# Autodesk Inventor assembly: BevelGear_Ref
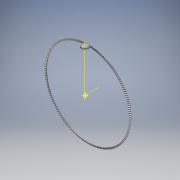
[picture p0: Inventor's stored thumbnail of the model, 180x180]
Saved by Autodesk Inventor 2017 (Build 210142000, 142)
## iProperties
Created: 2017-01-19
Part Number: BevelGear_Ref
Document SubType Name: Assembly
Designer: David Kopala
Author: David Kopala
## Documents named in this file (2)
- Z:\Documents\Drone\Drone\3D Models\Project\Chassis_04\BevelGear_Ref.iam
- Z:\Documents\Drone\Drone\3D Models\Project\Chassis_04\BevelGear_Ref\Design Accelerator\Bevel Gears3.iam
## Components (1 placed, 1 different names)
1. Bevel Gears:1 [sub-assembly]
## Named parameters: TEST = 25.4 mm
